# Autodesk Inventor assembly: F4C9-205 Bottom Bearing Block
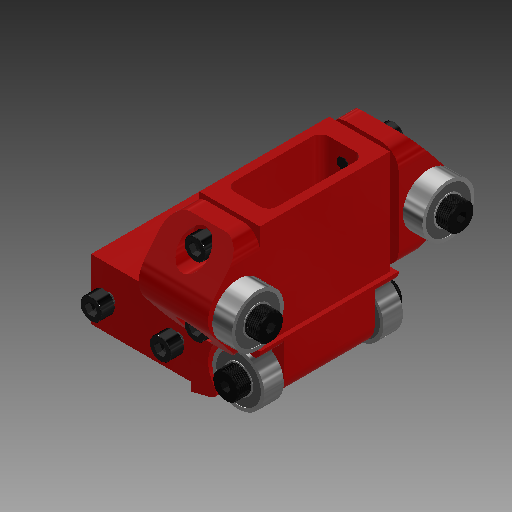
[picture p0: Inventor's stored thumbnail of the model, 512x512]
Saved by Autodesk Inventor 2021 (Build 250183000, 183)
## iProperties
Created: 2020-08-10
Part Number: F4C9-205 Bottom Bearing Block
Document SubType Name: Assembly
## Documents named in this file (12)
- C:\Users\Cal\Desktop\Robotics\Design\CollabPartsLib\Elevators\254 Blocks\254 Bottom Side Bearing Block.iam
- C:\Users\Cal\Desktop\Robotics\Design\CollabPartsLib\Power Transfer\Bearings\R4A.ipt
- E:\Middleton Robotics\Parts Library\Shaft Accessories\Bearings.ipt
- E:\Middleton Robotics\Parts Library\Hardware\Shoulder Bolt.ipt
- C:\Users\Cal\Desktop\Robotics\Design\CollabPartsLib\Hardware\Spacers & Standoffs\Aluminum Unthreaded Spacer (0.25in x 0.063Lg x 0.5OD).ipt
- E:\Middleton Robotics\Parts Library\Hardware\Spacers & Standoffs.ipt
- C:\Users\Cal\Desktop\Robotics\Design\CollabPartsLib\Hardware\Shoulder Bolt\0.25Dia x 0.75 Shoulder Bolt.ipt
- C:\Users\Cal\Desktop\Robotics\Design\CollabPartsLib\Hardware\Shoulder Bolt\0.25Dia x 0.5 Shoulder Bolt.ipt
- C:\Users\Cal\Desktop\Robotics\Design\CollabPartsLib\Elevators\254 Blocks\254 Side Bearing Block.ipt
- C:\Users\Cal\Desktop\Robotics\Design\CollabPartsLib\Elevators\254 Blocks\254 Bottom Bearing Block.ipt
- C:\Users\Cal\Desktop\Robotics\Design\CollabPartsLib\Hardware\Machine Screws\10-32 UNFx0.5625 Socket Head Cap Screw.ipt
- D:\FIRST\Design\CollabPartsLib\Hardware\Machine Screws.ipt
## Components (23 placed, 7 different names)
1. 254 Side Bearing Block:1 — Insert:11, Insert:12, Insert:24, Insert:27
2. R4A:1
3. 0.25Dia x 0.75 Shoulder Bolt:1
4. 254 Side Bearing Block:2 — Insert:13, Insert:14, Insert:28, Insert:29
5. R4A:2
6. 0.25Dia x 0.75 Shoulder Bolt:2
7. 254 Bottom Bearing Block:1 — Insert:11, Insert:12, Insert:13, Insert:14, Insert:20, Insert:23, Insert:25, Insert:26, Insert:30, Insert:31, Flush:1, Flush:2, Flush:3
8. Aluminum Unthreaded Spacer (0.25in x 0.063Lg x 0.5OD):1
9. Aluminum Unthreaded Spacer (0.25in x 0.063Lg x 0.5OD):2
10. Aluminum Unthreaded Spacer (0.25in x 0.063Lg x 0.5OD):5
11. R4A:6
12. 0.25Dia x 0.5 Shoulder Bolt:7 — Insert:20
13. Aluminum Unthreaded Spacer (0.25in x 0.063Lg x 0.5OD):6 — Insert:23
14. R4A:7
15. 0.25Dia x 0.5 Shoulder Bolt:8
16. 10-32 UNFx0.5625 Socket Head Cap Screw:9 — Insert:25
17. 10-32 UNFx0.5625 Socket Head Cap Screw:10 — Insert:26
18. 10-32 UNFx0.5625 Socket Head Cap Screw:11 — Insert:24
19. 10-32 UNFx0.5625 Socket Head Cap Screw:12 — Insert:27
20. 10-32 UNFx0.5625 Socket Head Cap Screw:13 — Insert:31
21. 10-32 UNFx0.5625 Socket Head Cap Screw:14 — Insert:30
22. 10-32 UNFx0.5625 Socket Head Cap Screw:15 — Insert:28
23. 10-32 UNFx0.5625 Socket Head Cap Screw:16 — Insert:29
## Relationships (27: Insert 24, Flush 3)
- [Insert]: R4A:1 ↔ 0.25Dia x 0.75 Shoulder Bolt:1
- [Insert] (1.5875 mm): 254 Side Bearing Block:1 ↔ R4A:1
- [Insert]: R4A:2 ↔ 0.25Dia x 0.75 Shoulder Bolt:2
- [Insert] (1.5875 mm): 254 Side Bearing Block:2 ↔ R4A:2
- [Insert]: 254 Side Bearing Block:1 ↔ Aluminum Unthreaded Spacer (0.25in x 0.063Lg x 0.5OD):1
- [Insert]: 254 Side Bearing Block:2 ↔ Aluminum Unthreaded Spacer (0.25in x 0.063Lg x 0.5OD):2
- Insert:11 (1.5875 mm): 254 Side Bearing Block:1 ↔ 254 Bottom Bearing Block:1
- Insert:12 (1.5875 mm): 254 Side Bearing Block:1 ↔ 254 Bottom Bearing Block:1
- Insert:13 (1.5875 mm): 254 Side Bearing Block:2 ↔ 254 Bottom Bearing Block:1
- Insert:14 (1.5875 mm): 254 Side Bearing Block:2 ↔ 254 Bottom Bearing Block:1
- [Insert]: R4A:6 ↔ 0.25Dia x 0.5 Shoulder Bolt:7
- [Insert]: Aluminum Unthreaded Spacer (0.25in x 0.063Lg x 0.5OD):5 ↔ R4A:6
- Insert:20: 254 Bottom Bearing Block:1 ↔ 0.25Dia x 0.5 Shoulder Bolt:7
- [Insert]: R4A:7 ↔ 0.25Dia x 0.5 Shoulder Bolt:8
- [Insert]: Aluminum Unthreaded Spacer (0.25in x 0.063Lg x 0.5OD):6 ↔ R4A:7
- Insert:23: 254 Bottom Bearing Block:1 ↔ Aluminum Unthreaded Spacer (0.25in x 0.063Lg x 0.5OD):6
- Insert:24: 254 Side Bearing Block:1 ↔ 10-32 UNFx0.5625 Socket Head Cap Screw:11
- Insert:25 (1.5875 mm): 254 Bottom Bearing Block:1 ↔ 10-32 UNFx0.5625 Socket Head Cap Screw:9
- Insert:26 (1.5875 mm): 254 Bottom Bearing Block:1 ↔ 10-32 UNFx0.5625 Socket Head Cap Screw:10
- Insert:27: 254 Side Bearing Block:1 ↔ 10-32 UNFx0.5625 Socket Head Cap Screw:12
- Insert:28: 254 Side Bearing Block:2 ↔ 10-32 UNFx0.5625 Socket Head Cap Screw:15
- Insert:29: 254 Side Bearing Block:2 ↔ 10-32 UNFx0.5625 Socket Head Cap Screw:16
- Insert:30 (1.5875 mm): 254 Bottom Bearing Block:1 ↔ 10-32 UNFx0.5625 Socket Head Cap Screw:14
- Insert:31 (1.5875 mm): 254 Bottom Bearing Block:1 ↔ 10-32 UNFx0.5625 Socket Head Cap Screw:13
- Flush:1: 254 Bottom Bearing Block:1
- Flush:2: 254 Bottom Bearing Block:1
- Flush:3: 254 Bottom Bearing Block:1
## Named parameters: d106_d77_d71 = 0 mm, d107_d78_d72 = 1.5875 mm, d108_d77_d71 = 0 mm, d109_d78_d72 = 1.5875 mm, d17_d14_d58_d106_d77_d71 = 0 mm, d18_d15 = 0 mm, d20_d17_d14_d58_d106_d77_d71 = 0 mm, d21_d18_d15 = 0 mm
